# Autodesk Inventor assembly: Desk Assembly
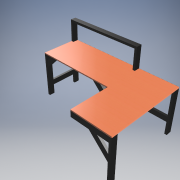
[picture p0: Inventor's stored thumbnail of the model, 180x180]
Saved by Autodesk Inventor 2018 (Build 220112000, 112)
## iProperties
Created: 2016-08-30
Part Number: Desk Assembly
Document SubType Name: Assembly
Designer: jjsch
Mass: 38826.1 g
Surface Area: 62997.1 cm^2
Volume: 68085.2 cm^3
Density: 0.570257 g/cm^3
Author: jjsch
## Documents named in this file (22)
- C:\Users\jjsch\Documents\Local\Engineering\EricsDesk\Desk Assembly.iam
- C:\Users\jjsch\Documents\Local\Engineering\EricsDesk\Pillar, Back.ipt
- C:\Users\jjsch\Documents\Local\Engineering\EricsDesk\Tabletop.ipt
- C:\Users\jjsch\Documents\Local\Engineering\EricsDesk\Joist, Side.ipt
- C:\Users\jjsch\Documents\Local\Engineering\EricsDesk\Pillar, Front.ipt
- C:\Users\jjsch\Documents\Local\Engineering\EricsDesk\Monitor Mount Bar.ipt
- C:\Users\jjsch\Documents\Local\Engineering\EricsDesk\Back Angle Piece.ipt
- C:\Users\jjsch\Documents\Local\Engineering\EricsDesk\Top Continuation Bar.ipt
- C:\Users\jjsch\Documents\Local\Engineering\EricsDesk\LTabletop.ipt
- C:\Users\jjsch\Documents\Local\Engineering\EricsDesk\LongColumn.ipt
- C:\Users\jjsch\Documents\Local\Engineering\EricsDesk\LSideBar.ipt
- C:\Users\jjsch\Documents\Local\Engineering\EricsDesk\AesteticTriangle.ipt
- C:\Users\jjsch\Documents\Local\Engineering\EricsDesk\L Extention Support Lower Piece.ipt
- C:\Users\jjsch\Documents\Local\Engineering\EricsDesk\FrontTriangularJoist.ipt
- C:\Users\jjsch\Documents\Local\Engineering\EricsDesk\FrontTriangularJoist_MIR.ipt
- C:\Users\jjsch\Documents\Local\Engineering\EricsDesk\L Support Joist.ipt
- C:\Users\jjsch\Documents\Local\Engineering\EricsDesk\Desk Assembly\AIP\FEA\c9kno9v34.fins
- C:\Users\jjsch\Documents\Local\Engineering\EricsDesk\Desk Assembly\AIP\FEA\c9kno9v34.fsat
- C:\Users\jjsch\Documents\Local\Engineering\EricsDesk\Desk Assembly\AIP\FEA\c9kno9v34.ftes
- C:\Users\jjsch\Documents\Local\Engineering\EricsDesk\Desk Assembly\AIP\FEA\c9kno9v34.fwiz
- C:\Users\jjsch\Documents\Local\Engineering\EricsDesk\Desk Assembly\AIP\FEA\c9kno9v4w.fmsh
- C:\Users\jjsch\Documents\Local\Engineering\EricsDesk\Desk Assembly\AIP\FEA\c9kno9v5s.fres
## Components (22 placed, 15 different names)
1. Pillar, Back:1 — Mate:3, Mate:4, Mate:5, Flush:1, Flush:3, Mate:13, Flush:7, Mate:41
2. Tabletop:1 — Mate:1, Mate:2, Mate:3, Mate:4, Mate:7, Mate:8, Mate:10, Mate:11, Flush:17, Mate:22, Mate:38, Flush:40, Mate:42, Flush:42, Mate:44, Flush:43
3. Pillar, Back:2 — Mate:1, Mate:2, Mate:6, Flush:2, Flush:4, Flush:8, Flush:9, Mate:14, Flush:25, Flush:36, Flush:37, Mate:43
4. Joist, Side:1 — Mate:6, Flush:2, Flush:4, Mate:8, Flush:6, Mate:12
5. Joist, Side:2 — Mate:5, Flush:1, Flush:3, Mate:7, Flush:5, Mate:9
6. Pillar, Front:1 — Mate:11, Flush:6, Mate:12, Flush:12, Flush:16, Mate:21, Symmetry:1
7. Pillar, Front:2 — Flush:5, Mate:9, Mate:10, Flush:10, Mate:15, Flush:11, Flush:39, Symmetry:1
8. Monitor Mount Bar:1 — Mate:13, Flush:7, Flush:8
9. Joist, Side:3 — Flush:9, Mate:14, Flush:12
10. Joist, Side:4 — Flush:10, Mate:15, Flush:11
11. Back Angle Piece:1 — Mate:41, Mate:42, Flush:42
12. Back Angle Piece:2 — Mate:43, Mate:44, Flush:43
13. Top Continuation Bar:1 — Flush:16, Mate:21, Flush:18, Flush:25
14. LTabletop:1 — Flush:17, Flush:18, Mate:22, Flush:20, Mate:23, Mate:24, Flush:21, Flush:22, Flush:26, Flush:29, Flush:30, Mate:31, Flush:33, Mate:37
15. LongColumn:1 — Mate:24, Flush:21, Flush:22, Flush:38
16. LongColumn:2 — Flush:20, Mate:23, Flush:26, Mate:39, Flush:41
17. LSideBar:1 — Flush:29, Flush:30, Mate:31, Flush:31, Flush:32, Mate:36, Mate:40
18. AesteticTriangle:1 — Flush:31, Flush:32, Flush:33, Mate:36, Mate:37
19. L Extention Support Lower Piece:1 — Flush:36, Flush:37, Flush:38
20. FrontTriangularJoist:1 — Flush:39, Mate:38, Flush:40
21. FrontTriangularJoist_MIR:1
22. L Support Joist:1 — Mate:39, Flush:41, Mate:40
## Relationships (63: Flush 33, Mate 29, Symmetry 1)
- Mate:1: Tabletop:1 ↔ Pillar, Back:2
- Mate:2: Tabletop:1 ↔ Pillar, Back:2
- Mate:3: Pillar, Back:1 ↔ Tabletop:1
- Mate:4: Pillar, Back:1 ↔ Tabletop:1
- Mate:5: Pillar, Back:1 ↔ Joist, Side:2
- Mate:6: Pillar, Back:2 ↔ Joist, Side:1
- Flush:1: Pillar, Back:1 ↔ Joist, Side:2
- Flush:2: Pillar, Back:2 ↔ Joist, Side:1
- Flush:3 (635 mm): Pillar, Back:1 ↔ Joist, Side:2
- Flush:4 (635 mm): Pillar, Back:2 ↔ Joist, Side:1
- Mate:7: Tabletop:1 ↔ Joist, Side:2
- Mate:8: Tabletop:1 ↔ Joist, Side:1
- Flush:5: Joist, Side:2 ↔ Pillar, Front:2
- Mate:9: Joist, Side:2 ↔ Pillar, Front:2
- Mate:10: Tabletop:1 ↔ Pillar, Front:2
- Mate:11: Tabletop:1 ↔ Pillar, Front:1
- Flush:6: Joist, Side:1 ↔ Pillar, Front:1
- Mate:12: Joist, Side:1 ↔ Pillar, Front:1
- Mate:13: Pillar, Back:1 ↔ Monitor Mount Bar:1
- Flush:7: Pillar, Back:1 ↔ Monitor Mount Bar:1
- Flush:8: Pillar, Back:2 ↔ Monitor Mount Bar:1
- Flush:9: Pillar, Back:2 ↔ Joist, Side:3
- Mate:14: Pillar, Back:2 ↔ Joist, Side:3
- Flush:10: Pillar, Front:2 ↔ Joist, Side:4
- Mate:15: Pillar, Front:2 ↔ Joist, Side:4
- Flush:11 (158.75 mm): Pillar, Front:2 ↔ Joist, Side:4
- Flush:12 (-158.75 mm): Pillar, Front:1 ↔ Joist, Side:3
- Flush:16: Pillar, Front:1 ↔ Top Continuation Bar:1
- Mate:21: Pillar, Front:1 ↔ Top Continuation Bar:1
- Flush:17: Tabletop:1 ↔ LTabletop:1
- Flush:18: Top Continuation Bar:1 ↔ LTabletop:1
- Mate:22: Tabletop:1 ↔ LTabletop:1
- Flush:20: LTabletop:1 ↔ LongColumn:2
- Mate:23: LTabletop:1 ↔ LongColumn:2
- Mate:24: LTabletop:1 ↔ LongColumn:1
- Flush:21: LTabletop:1 ↔ LongColumn:1
- Flush:22: LTabletop:1 ↔ LongColumn:1
- Flush:25: Pillar, Back:2 ↔ Top Continuation Bar:1
- Flush:26: LTabletop:1 ↔ LongColumn:2
- Flush:29: LTabletop:1 ↔ LSideBar:1
- Flush:30: LTabletop:1 ↔ LSideBar:1
- Mate:31: LTabletop:1 ↔ LSideBar:1
- Flush:31: LSideBar:1 ↔ AesteticTriangle:1
- Flush:32: LSideBar:1 ↔ AesteticTriangle:1
- Flush:33: LTabletop:1 ↔ AesteticTriangle:1
- Mate:36: LSideBar:1 ↔ AesteticTriangle:1
- Mate:37: LTabletop:1 ↔ AesteticTriangle:1
- Flush:36: Pillar, Back:2 ↔ L Extention Support Lower Piece:1
- Flush:37: Pillar, Back:2 ↔ L Extention Support Lower Piece:1
- Flush:38 (158.75 mm): LongColumn:1 ↔ L Extention Support Lower Piece:1
- Flush:39: Pillar, Front:2 ↔ FrontTriangularJoist:1
- Mate:38: Tabletop:1 ↔ FrontTriangularJoist:1
- Flush:40: Tabletop:1 ↔ FrontTriangularJoist:1
- Symmetry:1: Pillar, Front:1 ↔ Pillar, Front:2
- Mate:39: LongColumn:2 ↔ L Support Joist:1
- Flush:41: LongColumn:2 ↔ L Support Joist:1
- Mate:40: LSideBar:1 ↔ L Support Joist:1
- Mate:41: Pillar, Back:1 ↔ Back Angle Piece:1
- Mate:42: Tabletop:1 ↔ Back Angle Piece:1
- Flush:42: Tabletop:1 ↔ Back Angle Piece:1
- Mate:43: Pillar, Back:2 ↔ Back Angle Piece:2
- Mate:44: Tabletop:1 ↔ Back Angle Piece:2
- Flush:43: Tabletop:1 ↔ Back Angle Piece:2
## Named parameters: sa_0 = 133447
note: some values were not read from the file. Shown as the stored number, unit unknown: "sa_0".
